# Autodesk Inventor assembly: HSMCS50-N
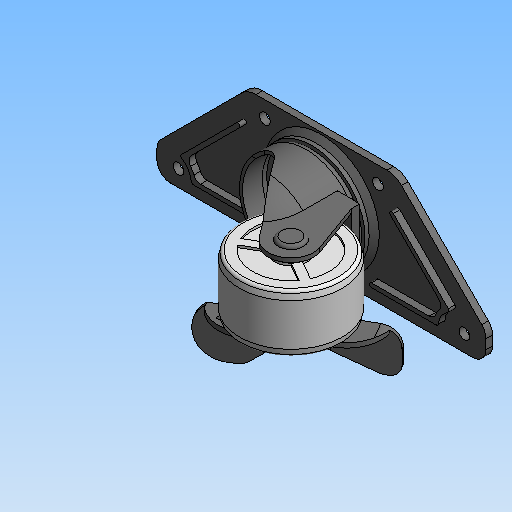
[picture p0: Inventor's stored thumbnail of the model, 512x512]
Saved by Autodesk Inventor 2020 (Build 240168000, 168)
## iProperties
Part Number: HSMCS50-N
Catalog Web Link: www.cadenas.de
Description: HSMCS-Casters for Aluminum Frame Swivel Type with Stopper
Vendor: MISUMI
Document SubType Name: Assembly
Designer: partserver
Manufacturer: MISUMI
Mass: 97.2703 g
Surface Area: 455.243 cm^2
Volume: 97.2703 cm^3
Density: 1 g/cm^3
Category: PARTsolutions
Company: MISUMI
PSOL_IDENT_0: {$CADENAS_DATA\23d-libs\misumi\metric\39_accessories_for_al_extrusions\hsmcs_asmtab.prj},166 {VTYP=3
PSOL_IDENT_1: D},{STYP=ASSTAB},{NB=HSMCS50-N},{LINA=HSMCS50-N},{NN=HSMCS},{DATE=30.06.2021 13:18:54},{GEOMDATE=31.
PSOL_IDENT_2: 08.2009},{VERSION=},{LINEID=10},{WBVAR=MATW},{WBNUMERIC=}  {NB=HSMCS50-N},{LINA=HSMCS50-N},{KT=DUMMY
PSOL_IDENT_3: },{PN=HSMCS50-N},{TS=HSMCS},{MATB=SPHC(Low Carbon Steel)(1.0330_DC01(St.12)or 1.0320_St.22)},{STB=Tr
PSOL_IDENT_4: ivalent Chromate Plating},{MATW=N},{MATW1='R','Synthetic Rubber','N','Nylon'},{BSP=Available},{BWP=N
PSOL_IDENT_5: one},{D=50},{AF=HFS5-2020},{H=70},{B=28},{DD=5.3},{E=27},{RR=67},{MASS=496},{AL=600},{DD1=34.703},{D
PSOL_IDENT_6: D2=2.800},{DD3=56.000},{DD4=29.936},{DD5=42.809},{DD6=12.029},{DD7=37},{DD8=27.000},{DD9=22.000},{DD
PSOL_IDENT_7: 10=45.000},{DD11=30.233},{COLOR=1.00,1.00,1.00,0.00},{PPATH=../../../misumi/metric/39_accessories_fo
PSOL_IDENT_8: r_al_extrusions/hsmc_asmtpl.prj}
NB: HSMCS50-N
NN: HSMCS
NT: Casters for Aluminum Frame Swivel Type with Stopper
NBSYN: $PN.
LINA: HSMCS50-N
CATALOG: Misumi
PN: HSMCS50-N
MATB: Low Carbon Steel
STB: Trivalent Chromate Plating
MATW: Nylon
BSP: Provided
BWP: Not Provided
D: 50
AF: HFS5-2020
H: 70
B: 28
DD: 5.3
E: 27
RR: 67
MASS: 496
AL: 600
SUPPLIER: MISUMI
ARTICLENO: HSMCS50-N
BOMINFO: HSMCS50-N
CREATOR: CADENAS GmbH
Title: HSMCS50-N
Author: Cadenas PARTsolutions
Comments: Casters for Aluminum Frame Swivel Type with Stopper
## Documents named in this file (6)
- C:\Users\lvglv\Documents\GitHub\Eto_Project\Hardware\Parts\MISUMI\HSMCS50-N_Autodesk_Inventor_2020_20210712\AIS2020\HSMCS50-N.iam
- C:\Users\lvglv\Documents\GitHub\Eto_Project\Hardware\Parts\MISUMI\HSMCS50-N_Autodesk_Inventor_2020_20210712\AIS2020\DUMMY-HSMCS50-N.ipt
- C:\Users\lvglv\Documents\GitHub\Eto_Project\Hardware\Parts\MISUMI\HSMCS50-N_Autodesk_Inventor_2020_20210712\AIS2020\SWIVEL-HSMCS50.ipt
- C:\Users\lvglv\Documents\GitHub\Eto_Project\Hardware\Parts\MISUMI\HSMCS50-N_Autodesk_Inventor_2020_20210712\AIS2020\BODY-HSMCS50.ipt
- C:\Users\lvglv\Documents\GitHub\Eto_Project\Hardware\Parts\MISUMI\HSMCS50-N_Autodesk_Inventor_2020_20210712\AIS2020\WHEEL-HSMCS50-N.ipt
- C:\Users\lvglv\Documents\GitHub\Eto_Project\Hardware\Parts\MISUMI\HSMCS50-N_Autodesk_Inventor_2020_20210712\AIS2020\STOPPER-HSMCS50.ipt
## Components (5 placed, 5 different names)
1. DUMMY-HSMCS50-N:1 — dummy_to_swivel_XY@1 <-> swivel_to_dummy_XY@2, dummy_to_swivel_Z@1 <-> swivel_to_dummy_Z@2, dummy_to_swivel_YZ@1 <-> swivel_to_dummy_YZ@2
2. SWIVEL-HSMCS50:1 — dummy_to_swivel_XY@1 <-> swivel_to_dummy_XY@2, dummy_to_swivel_Z@1 <-> swivel_to_dummy_Z@2, dummy_to_swivel_YZ@1 <-> swivel_to_dummy_YZ@2, swivel_to_body_XY@2 <-> body_to_swivel_XY@3, swivel_to_body_Z@2 <-> body_to_swivel_Z@3
3. BODY-HSMCS50:1 — swivel_to_body_XY@2 <-> body_to_swivel_XY@3, swivel_to_body_Z@2 <-> body_to_swivel_Z@3, body_to_wheel_XY@3 <-> wheel_to_body_XY@4, body_to_wheel_Z@3 <-> wheel_to_body_Z@4, body_to_stopper_right_XY@3 <-> stopper_to_body_XY@5, body_to_stopper_right_Z@3 <-> stopper_to_body_Z@5
4. WHEEL-HSMCS50-N:1 — body_to_wheel_XY@3 <-> wheel_to_body_XY@4, body_to_wheel_Z@3 <-> wheel_to_body_Z@4
5. STOPPER-HSMCS50:1 — body_to_stopper_right_XY@3 <-> stopper_to_body_XY@5, body_to_stopper_right_Z@3 <-> stopper_to_body_Z@5
## Relationships (9: Mate 7, Angle 1, Flush 1)
- dummy_to_swivel_XY@1 <-> swivel_to_dummy_XY@2 [Mate]: DUMMY-HSMCS50-N:1 ↔ SWIVEL-HSMCS50:1
- dummy_to_swivel_Z@1 <-> swivel_to_dummy_Z@2 [Mate]: DUMMY-HSMCS50-N:1 ↔ SWIVEL-HSMCS50:1
- dummy_to_swivel_YZ@1 <-> swivel_to_dummy_YZ@2 [Angle] (0 deg): DUMMY-HSMCS50-N:1 ↔ SWIVEL-HSMCS50:1
- swivel_to_body_XY@2 <-> body_to_swivel_XY@3 [Mate] (3.2 mm): SWIVEL-HSMCS50:1 ↔ BODY-HSMCS50:1
- swivel_to_body_Z@2 <-> body_to_swivel_Z@3 [Mate]: SWIVEL-HSMCS50:1 ↔ BODY-HSMCS50:1
- body_to_wheel_XY@3 <-> wheel_to_body_XY@4 [Mate]: BODY-HSMCS50:1 ↔ WHEEL-HSMCS50-N:1
- body_to_wheel_Z@3 <-> wheel_to_body_Z@4 [Mate]: BODY-HSMCS50:1 ↔ WHEEL-HSMCS50-N:1
- body_to_stopper_right_XY@3 <-> stopper_to_body_XY@5 [Flush]: BODY-HSMCS50:1 ↔ STOPPER-HSMCS50:1
- body_to_stopper_right_Z@3 <-> stopper_to_body_Z@5 [Mate]: BODY-HSMCS50:1 ↔ STOPPER-HSMCS50:1
